# Autodesk Inventor assembly: DriveTrain
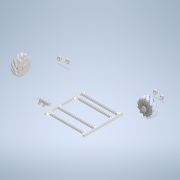
[picture p0: Inventor's stored thumbnail of the model, 180x180]
Saved by Autodesk Inventor 2020.2 (Build 242310000, 310)
## iProperties
Created: 2020-01-29
Part Number: DriveTrain
Document SubType Name: Assembly
Designer: yukin
Author: yukin
## Documents named in this file (14)
- C:\Users\AOFUser\Documents\GitHub\CAD\Robotics 2019-2020\Assembly\DriveTrain\DriveTrain.iam
- C:\Users\AOFUser\Documents\GitHub\CAD\Robotics 2019-2020\Assembly\DriveTrain\RevHexMotor\RevHexMotor.iam
- C:\Users\AOFUser\Documents\GitHub\CAD\Robotics 2019-2020\Assembly\DriveTrain\MotorMount_vCAD.ipt
- C:\Users\AOFUser\Documents\GitHub\CAD\Robotics 2019-2020\Assembly\DriveTrain\Extrusions\17in.ipt
- C:\Users\AOFUser\Documents\GitHub\CAD\Robotics 2019-2020\Assembly\DriveTrain\CornerBracket.ipt
- C:\Users\AOFUser\Documents\GitHub\CAD\Robotics 2019-2020\Assembly\DriveTrain\MotorMountBackSide.ipt
- C:\Users\AOFUser\Documents\GitHub\CAD\Robotics 2019-2020\Assembly\DriveTrain\Extrusions\18in.ipt
- C:\Users\AOFUser\Documents\GitHub\CAD\Robotics 2019-2020\Assembly\DriveTrain\BearingHolder.ipt
- C:\Users\AOFUser\Documents\GitHub\CAD\Robotics 2019-2020\Assembly\DriveTrain\LMecaWheel\LMecaWheel.iam
- C:\Users\AOFUser\Documents\GitHub\CAD\Robotics 2019-2020\Assembly\DriveTrain\RMecaWheel\RMecaWheel.iam
- C:\Users\AOFUser\Documents\GitHub\CAD\Robotics 2019-2020\Assembly\DriveTrain\HexHub.ipt
- C:\Users\AOFUser\Documents\GitHub\CAD\Robotics 2019-2020\Assembly\DriveTrain\WheelMount_v1_vCAD.ipt
- C:\Users\AOFUser\Documents\GitHub\CAD\Robotics 2019-2020\Assembly\DriveTrain\WheelMount_v2_vCAD.ipt
- C:\Users\AOFUser\Documents\GitHub\CAD\Robotics 2019-2020\Assembly\DriveTrain\HexShaft.ipt
## Components (39 placed, 13 different names)
1. RevHexMotor:1 [sub-assembly] — Rotational:1, Insert:1
2. MotorMount_vCAD:1 — Rotational:1, Flush:21
3. 17in:1 — Mate:1, Flush:1, Flush:2, Flush:12, Flush:13, Mate:7, Mate:8, Flush:14, Flush:15, Mate:11, Flush:19
4. 17in:2 — Flush:3, Mate:2, Flush:4, Flush:8, Flush:9, Mate:5, Flush:10, Mate:6, Flush:11, Mate:12, Flush:28
5. CornerBracket:1 — Flush:3, Mate:2, Flush:4, Flush:24, Mate:14
6. CornerBracket:2 — Mate:1, Flush:1, Flush:2, Flush:22, Flush:23, Mate:13
7. CornerBracket:3 — Mate:8, Flush:14, Flush:15
8. CornerBracket:4 — Flush:12, Flush:13, Mate:7
9. CornerBracket:5 — Flush:8, Flush:9, Mate:5
10. CornerBracket:6 — Flush:10, Mate:6, Flush:11
11. CornerBracket:7 — Mate:11, Flush:19, Flush:25, Mate:15, Flush:26
12. CornerBracket:8 — Mate:12, Flush:27, Mate:16, Flush:28
13. MotorMountBackSide:1 — Insert:1, Flush:21
14. 18in:1 — Flush:25, Mate:15, Flush:26, Flush:27, Mate:16, Flush:29, Flush:30, Mate:17, Flush:31, Mate:18
15. 18in:2 — Flush:22, Flush:23, Mate:13, Flush:24, Mate:14, Flush:32, Mate:19, Flush:33, Mate:20, Flush:34, Flush:37
16. CornerBracket:9 — Flush:32, Mate:19, Flush:33, Mate:23, Flush:38
17. CornerBracket:10 — Mate:20, Flush:34, Mate:22
18. CornerBracket:11 — Flush:29, Flush:30, Mate:17
19. CornerBracket:12 — Flush:31, Mate:18, Flush:35, Mate:21, Flush:36
20. 17in:3 — Flush:35, Mate:21, Flush:36, Mate:22, Flush:39, Flush:40, Mate:24, Flush:43, Flush:44, Mate:26
21. 17in:4 — Mate:23, Flush:37, Flush:38, Mate:25, Flush:41, Flush:42, Flush:45, Flush:46, Mate:27
22. CornerBracket:13 — Flush:39, Flush:40, Mate:24
23. CornerBracket:14 — Flush:43, Flush:44, Mate:26
24. CornerBracket:15 — Mate:25, Flush:41, Flush:42
25. CornerBracket:16 — Flush:45, Flush:46, Mate:27
26. BearingHolder:1
27. BearingHolder:2
28. BearingHolder:3
29. BearingHolder:4
30. LMecaWheel:2 [sub-assembly] — Insert:10, Insert:11, Insert:12, Insert:13
31. RMecaWheel:1 [sub-assembly] — Insert:2, Insert:3, Insert:6, Insert:7
32. HexHub:2 — Insert:8, Insert:9
33. HexHub:3 — Insert:4, Insert:5
34. WheelMount_v1_vCAD:1 — Insert:12, Insert:13
35. WheelMount_v1_vCAD:2 — Insert:6, Insert:7
36. WheelMount_v2_vCAD:1 — Insert:2, Insert:3, Insert:4, Insert:5
37. HexShaft:1
38. HexShaft:2
39. WheelMount_v2_vCAD:2 — Insert:8, Insert:9, Insert:10, Insert:11
## Relationships (76: Flush 39, Mate 23, Insert 13, RevoluteJoint 1)
- Rotational:1 [RevoluteJoint]: RevHexMotor:1 ↔ MotorMount_vCAD:1
- Mate:1: 17in:1 ↔ CornerBracket:2
- Flush:1: 17in:1 ↔ CornerBracket:2
- Flush:2: 17in:1 ↔ CornerBracket:2
- Flush:3: 17in:2 ↔ CornerBracket:1
- Mate:2: 17in:2 ↔ CornerBracket:1
- Flush:4: 17in:2 ↔ CornerBracket:1
- Flush:8: 17in:2 ↔ CornerBracket:5
- Flush:9: 17in:2 ↔ CornerBracket:5
- Mate:5: 17in:2 ↔ CornerBracket:5
- Flush:10: 17in:2 ↔ CornerBracket:6
- Mate:6: 17in:2 ↔ CornerBracket:6
- Flush:11: 17in:2 ↔ CornerBracket:6
- Flush:12: 17in:1 ↔ CornerBracket:4
- Flush:13: 17in:1 ↔ CornerBracket:4
- Mate:7: 17in:1 ↔ CornerBracket:4
- Mate:8: 17in:1 ↔ CornerBracket:3
- Flush:14: 17in:1 ↔ CornerBracket:3
- Flush:15: 17in:1 ↔ CornerBracket:3
- Mate:11: 17in:1 ↔ CornerBracket:7
- Flush:19: 17in:1 ↔ CornerBracket:7
- Mate:12: 17in:2 ↔ CornerBracket:8
- Insert:1: RevHexMotor:1 ↔ MotorMountBackSide:1
- Flush:21: MotorMount_vCAD:1 ↔ MotorMountBackSide:1
- Flush:22: CornerBracket:2 ↔ 18in:2
- Flush:23: CornerBracket:2 ↔ 18in:2
- Mate:13: CornerBracket:2 ↔ 18in:2
- Flush:24: CornerBracket:1 ↔ 18in:2
- Mate:14: CornerBracket:1 ↔ 18in:2
- Flush:25: CornerBracket:7 ↔ 18in:1
- Mate:15: CornerBracket:7 ↔ 18in:1
- Flush:26: CornerBracket:7 ↔ 18in:1
- Flush:27: CornerBracket:8 ↔ 18in:1
- Mate:16: CornerBracket:8 ↔ 18in:1
- Flush:28: 17in:2 ↔ CornerBracket:8
- Flush:29: 18in:1 ↔ CornerBracket:11
- Flush:30: 18in:1 ↔ CornerBracket:11
- Mate:17: 18in:1 ↔ CornerBracket:11
- Flush:31: 18in:1 ↔ CornerBracket:12
- Mate:18: 18in:1 ↔ CornerBracket:12
- Flush:32: 18in:2 ↔ CornerBracket:9
- Mate:19: 18in:2 ↔ CornerBracket:9
- Flush:33: 18in:2 ↔ CornerBracket:9
- Mate:20: 18in:2 ↔ CornerBracket:10
- Flush:34: 18in:2 ↔ CornerBracket:10
- Flush:35: CornerBracket:12 ↔ 17in:3
- Mate:21: CornerBracket:12 ↔ 17in:3
- Flush:36: CornerBracket:12 ↔ 17in:3
- Mate:22: CornerBracket:10 ↔ 17in:3
- Mate:23: CornerBracket:9 ↔ 17in:4
- Flush:37: 18in:2 ↔ 17in:4
- Flush:38: CornerBracket:9 ↔ 17in:4
- Flush:39: 17in:3 ↔ CornerBracket:13
- Flush:40: 17in:3 ↔ CornerBracket:13
- Mate:24: 17in:3 ↔ CornerBracket:13
- Mate:25: 17in:4 ↔ CornerBracket:15
- Flush:41: 17in:4 ↔ CornerBracket:15
- Flush:42: 17in:4 ↔ CornerBracket:15
- Flush:43: 17in:3 ↔ CornerBracket:14
- Flush:44: 17in:3 ↔ CornerBracket:14
- Mate:26: 17in:3 ↔ CornerBracket:14
- Flush:45: 17in:4 ↔ CornerBracket:16
- Flush:46: 17in:4 ↔ CornerBracket:16
- Mate:27: 17in:4 ↔ CornerBracket:16
- Insert:2: RMecaWheel:1 ↔ WheelMount_v2_vCAD:1
- Insert:3: RMecaWheel:1 ↔ WheelMount_v2_vCAD:1
- Insert:4: HexHub:3 ↔ WheelMount_v2_vCAD:1
- Insert:5: HexHub:3 ↔ WheelMount_v2_vCAD:1
- Insert:6: RMecaWheel:1 ↔ WheelMount_v1_vCAD:2
- Insert:7: RMecaWheel:1 ↔ WheelMount_v1_vCAD:2
- Insert:8: HexHub:2 ↔ WheelMount_v2_vCAD:2
- Insert:9: HexHub:2 ↔ WheelMount_v2_vCAD:2
- Insert:10: LMecaWheel:2 ↔ WheelMount_v2_vCAD:2
- Insert:11: LMecaWheel:2 ↔ WheelMount_v2_vCAD:2
- Insert:12: LMecaWheel:2 ↔ WheelMount_v1_vCAD:1
- Insert:13: LMecaWheel:2 ↔ WheelMount_v1_vCAD:1
